# Autodesk Inventor assembly: claw
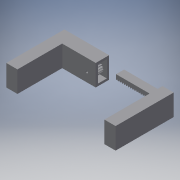
[picture p0: Inventor's stored thumbnail of the model, 180x180]
Saved by Autodesk Inventor 2019 (Build 230136000, 136)
## iProperties
Created: 2018-11-15
Part Number: claw
Document SubType Name: Assembly
Designer: Charlie
Author: Charlie
## Documents named in this file (4)
- F:\school\senior\fall\senior_design\claw\claw.iam
- F:\school\senior\fall\senior_design\claw\hollowPart.ipt
- F:\school\senior\fall\senior_design\claw\rackPart.ipt
- F:\school\senior\fall\senior_design\claw\gear.ipt
## Components (3 placed, 3 different names)
1. hollowPart:1 — Mate:1, Flush:1, Flush:2, Mate:2
2. rackPart:1 — Flush:1, Flush:2
3. gear:1 — Mate:1, Mate:2
## Relationships (4: Mate 2, Flush 2)
- Mate:1: hollowPart:1 ↔ gear:1
- Flush:1: hollowPart:1 ↔ rackPart:1
- Flush:2: hollowPart:1 ↔ rackPart:1
- Mate:2 (0.254 mm): hollowPart:1 ↔ gear:1
